# Autodesk Inventor assembly: Mass 1 Group
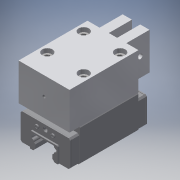
[picture p0: Inventor's stored thumbnail of the model, 180x180]
Saved by Autodesk Inventor 2016 (Build 200138000, 138)
## iProperties
Created: 2015-07-07
Part Number: Mass 1 Group
Document SubType Name: Assembly
Designer: Dennis
Mass: 2344.9 g
Surface Area: 738.737 cm^2
Volume: 504.146 cm^3
Density: 4.65123 g/cm^3
Author: Dennis
## Documents named in this file (4)
- C:\Users\Jason\Dropbox\NI Work\NI Ball Bearing Slider Crank\CAD\Assemblies\Mass 1 Group.iam
- C:\Users\Jason\Dropbox\NI Work\NI Ball Bearing Slider Crank\CAD\McMaster Parts\Ball Bearing Carriage - Ball-Bearing Carriage, Threaded-Hole, for 34 mm Rail Width - 6709K21.ipt
- C:\Users\Jason\Dropbox\NI Work\NI Ball Bearing Slider Crank\CAD\Mass 1 V2.ipt
- C:\Users\Jason\Dropbox\NI Work\NI Ball Bearing Slider Crank\CAD\McMaster Parts\M8x1.25x50.ipt
## Components (6 placed, 3 different names)
1. Ball Bearing Carriage - Ball-Bearing Carriage, Threaded-Hole, for 34 mm Rail Width - 6709K21:1 — Mate:9, Mate:10, Mate:11
2. Mass 1 V2:1 — Mate:9, Mate:10, Mate:11, Mate:12, Mate:13, Mate:14, Mate:15, Mate:16, Mate:17, Mate:18, Mate:19
3. M8x1.25x50:1 — Mate:12, Mate:16
4. M8x1.25x50:2 — Mate:13, Mate:17
5. M8x1.25x50:3 — Mate:14, Mate:18
6. M8x1.25x50:4 — Mate:15, Mate:19
## Relationships (11: Mate 11)
- Mate:9: Ball Bearing Carriage - Ball-Bearing Carriage, Threaded-Hole, for 34 mm Rail Width - 6709K21:1 ↔ Mass 1 V2:1
- Mate:10: Ball Bearing Carriage - Ball-Bearing Carriage, Threaded-Hole, for 34 mm Rail Width - 6709K21:1 ↔ Mass 1 V2:1
- Mate:11: Ball Bearing Carriage - Ball-Bearing Carriage, Threaded-Hole, for 34 mm Rail Width - 6709K21:1 ↔ Mass 1 V2:1
- Mate:12: Mass 1 V2:1 ↔ M8x1.25x50:1
- Mate:13: Mass 1 V2:1 ↔ M8x1.25x50:2
- Mate:14: Mass 1 V2:1 ↔ M8x1.25x50:3
- Mate:15: Mass 1 V2:1 ↔ M8x1.25x50:4
- Mate:16: Mass 1 V2:1 ↔ M8x1.25x50:1
- Mate:17: Mass 1 V2:1 ↔ M8x1.25x50:2
- Mate:18: Mass 1 V2:1 ↔ M8x1.25x50:3
- Mate:19: Mass 1 V2:1 ↔ M8x1.25x50:4
